# Autodesk Inventor assembly: ExternalMotorizedOuterRingAssembly
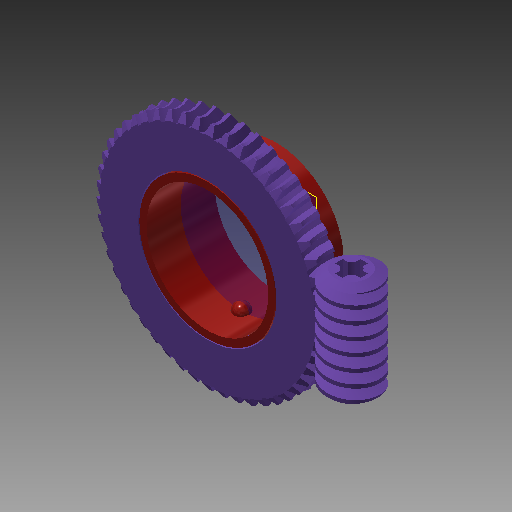
[picture p0: Inventor's stored thumbnail of the model, 512x512]
Saved by Autodesk Inventor 2019.3 (Build 233278000, 278)
## iProperties
Created: 2018-12-30
Part Number: ExternalMotorizedOuterRingAssembly
Document SubType Name: Assembly
Designer: steele
Author: steele
## Documents named in this file (3)
- C:\git\CAD-Development\robSteele\ShapeWays\TelescopeProjects\Focuser\ExternalMotorizedOuterRingAssembly.iam
- C:\git\CAD-Development\robSteele\ShapeWays\TelescopeProjects\Focuser\ExternalMotorizedOuterRing.ipt
- C:\git\CAD-Development\robSteele\ShapeWays\TelescopeProjects\Focuser\ExternalMotorizedOuterRingAssembly\Design Accelerator\Worm Gears8.iam
## Components (2 placed, 2 different names)
1. Worm Gears:1 [sub-assembly] — Insert:1, Angle:1
2. ExternalMotorizedOuterRing:1 — Insert:1
## Relationships (2: Insert 1, Angle 1)
- Insert:1: Worm Gears:1 ↔ ExternalMotorizedOuterRing:1
- Angle:1 (0 deg): Worm Gears:1
